# Autodesk Inventor assembly: Base
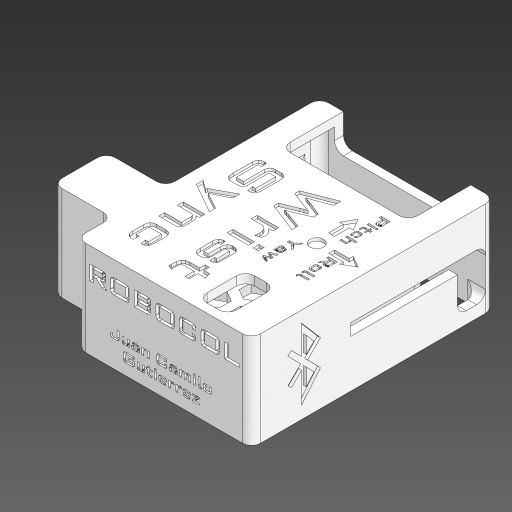
[picture p0: Inventor's stored thumbnail of the model, 512x512]
Saved by Autodesk Inventor 2023.3 (Build 273359000, 359)
## iProperties
Created: 2023-04-15
Part Number: Base
Document SubType Name: Assembly
Designer: jcgg2
Mass: 90.2386 g
Surface Area: 484.337 cm^2
Volume: 90.2386 cm^3
Density: 1 g/cm^3
Author: jcgg2
## Documents named in this file (4)
- F:\OneDrive\U\2023-10\Tesis IELE\Final version\Base.iam
- F:\OneDrive\U\2023-10\Tesis IELE\Final version\PCB base.ipt
- F:\OneDrive\U\2023-10\Tesis IELE\Final version\Hand.ipt
- F:\OneDrive\U\2023-10\Tesis IELE\Final version\Carcasa.ipt
## Components (3 placed, 3 different names)
1. PCB base:1 — Mate:1, Mate:2, Mate:3
2. Hand:1
3. Carcasa:1 — Mate:1, Mate:2, Mate:3
## Relationships (3: Mate 3)
- Mate:1: PCB base:1 ↔ Carcasa:1
- Mate:2: PCB base:1 ↔ Carcasa:1
- Mate:3 (2 mm): PCB base:1 ↔ Carcasa:1
